# Autodesk Inventor assembly: CORTADORA_RECTA
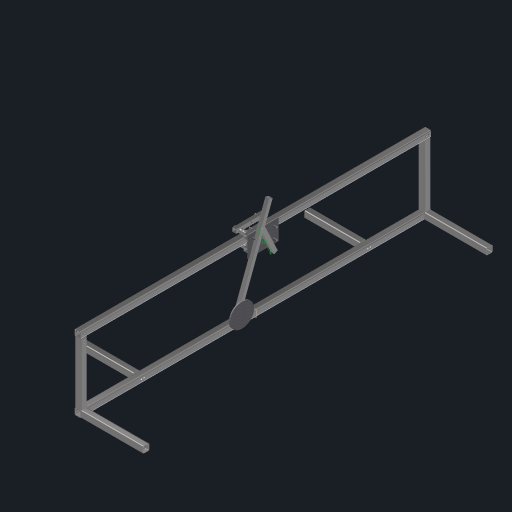
[picture p0: Inventor's stored thumbnail of the model, 512x512]
Saved by Autodesk Inventor 2024.3 (Build 283343000, 343)
## iProperties
_SolveAssemblyDoc: Frame Generator Solve Assembly
_Version: 25.0.0
Created: 2024-05-30
Part Number: CORTADORA_RECTA
Material: Generic
Document SubType Name: Assembly
Designer: Niler
Author: Niler
## Documents named in this file (10)
- C:\Users\Niler\OneDrive\Escritorio\RECICLADOR\RECICLADOR_MODELO_3D\CORTADORA_RECTA_2M\CORTADORA_RECTA.iam
- C:\Users\Niler\OneDrive\Escritorio\RECICLADOR\RECICLADOR_MODELO_3D\CORTADORA_RECTA_2M\ESQUELETO_CORTADORA_RECTA.ipt
- C:\Users\Niler\OneDrive\Escritorio\RECICLADOR\RECICLADOR_MODELO_3D\CORTADORA_RECTA_2M\CORTADORA_RECTA\Frame\Frame 1717303402985.iam
- C:\Users\Niler\OneDrive\Escritorio\RECICLADOR\RECICLADOR_MODELO_3D\CORTADORA_RECTA_2M\ACOPLE_TORNILLO_DOBLE.ipt
- C:\Users\Niler\OneDrive\Escritorio\RECICLADOR\RECICLADOR_MODELO_3D\LIBRERIA\en-US\AS 1112 (2)\AS 1112 - M8  Type 5.ipt
- C:\Users\Niler\OneDrive\Escritorio\RECICLADOR\RECICLADOR_MODELO_3D\LIBRERIA\en-US\AS 1110\AS 1110 - M6 x 12.ipt
- C:\Users\Niler\OneDrive\Escritorio\RECICLADOR\RECICLADOR_MODELO_3D\CORTADORA_RECTA_2M\CARRITO.iam
- C:\Users\Niler\OneDrive\Escritorio\RECICLADOR\RECICLADOR_MODELO_3D\CORTADORA_RECTA_2M\BRAZO_CARRITO.iam
- C:\Users\Niler\OneDrive\Escritorio\RECICLADOR\RECICLADOR_MODELO_3D\CORTADORA_RECTA_2M\DISCO.ipt
- C:\Users\Niler\OneDrive\Escritorio\RECICLADOR\RECICLADOR_MODELO_3D\CORTADORA_RECTA_2M\BRAZO_CARRITO_V2.iam
## Components (14 placed, 9 different names)
1. ESQUELETO_CORTADORA_RECTA:1
2. Frame 1717303402985:1 [sub-assembly] — Mate:1, Mate:2, Mate:3, Insert:3, Insert:4, Insert:5, Insert:6, Tangent:1, Tangent:2, Tangent:3
3. ACOPLE_TORNILLO_DOBLE:1 — Insert:1, Insert:2, Mate:1, Mate:2, Mate:3
4. AS 1112 (2) - Metric M8  Type 5:1 — Insert:1
5. AS 1112 (2) - Metric M8  Type 5:2 — Insert:2
6. AS 1110 - Metric M6 x 12:1 — Insert:3
7. AS 1110 - Metric M6 x 12:2 — Insert:4
8. AS 1110 - Metric M6 x 12:3 — Insert:5
9. AS 1110 - Metric M6 x 12:4 — Insert:6
10. CARRITO:1 [sub-assembly] — Tangent:1, Tangent:2, Mate:4, Tangent:3, Mate:5, Mate:8, Mate:9, Mate:10
11. BRAZO_CARRITO:1 [sub-assembly] — Mate:4, Mate:5, Mate:6, Mate:7
12. DISCO:1 — Mate:6, Mate:7
13. BRAZO_CARRITO_V2:1 [sub-assembly] — Mate:8, Mate:9, Mate:10, Mate:11, Mate:12
14. DISCO:2 — Mate:11, Mate:12
## Relationships (21: Mate 12, Insert 6, Tangent 3)
- Insert:1: ACOPLE_TORNILLO_DOBLE:1 ↔ AS 1112 (2) - Metric M8  Type 5:1
- Insert:2: ACOPLE_TORNILLO_DOBLE:1 ↔ AS 1112 (2) - Metric M8  Type 5:2
- Mate:1 (-20 mm): Frame 1717303402985:1 ↔ ACOPLE_TORNILLO_DOBLE:1
- Mate:2: Frame 1717303402985:1 ↔ ACOPLE_TORNILLO_DOBLE:1
- Mate:3: Frame 1717303402985:1 ↔ ACOPLE_TORNILLO_DOBLE:1
- Insert:3: Frame 1717303402985:1 ↔ AS 1110 - Metric M6 x 12:1
- Insert:4: Frame 1717303402985:1 ↔ AS 1110 - Metric M6 x 12:2
- Insert:5: Frame 1717303402985:1 ↔ AS 1110 - Metric M6 x 12:3
- Insert:6: Frame 1717303402985:1 ↔ AS 1110 - Metric M6 x 12:4
- Tangent:1: Frame 1717303402985:1 ↔ CARRITO:1
- Tangent:2: Frame 1717303402985:1 ↔ CARRITO:1
- Mate:4: CARRITO:1 ↔ BRAZO_CARRITO:1
- Tangent:3: Frame 1717303402985:1 ↔ CARRITO:1
- Mate:5: CARRITO:1 ↔ BRAZO_CARRITO:1
- Mate:6: BRAZO_CARRITO:1 ↔ DISCO:1
- Mate:7: BRAZO_CARRITO:1 ↔ DISCO:1
- Mate:8: CARRITO:1 ↔ BRAZO_CARRITO_V2:1
- Mate:9: CARRITO:1 ↔ BRAZO_CARRITO_V2:1
- Mate:10: CARRITO:1 ↔ BRAZO_CARRITO_V2:1
- Mate:11: BRAZO_CARRITO_V2:1 ↔ DISCO:2
- Mate:12: BRAZO_CARRITO_V2:1 ↔ DISCO:2
